# Autodesk Inventor assembly: Assembly5
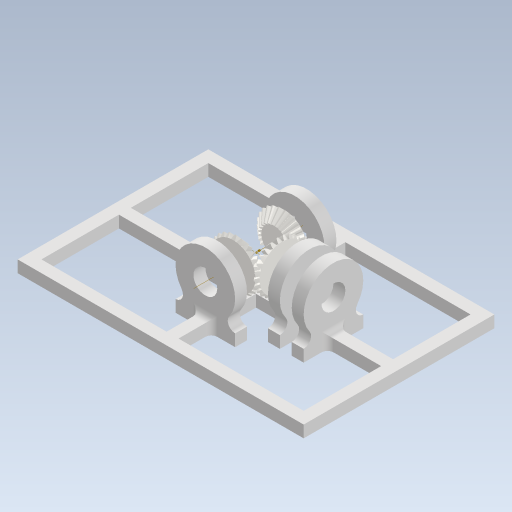
[picture p0: Inventor's stored thumbnail of the model, 512x512]
Saved by Autodesk Inventor 2023 (Build 270158000, 158)
## iProperties
Created: 2023-02-24
Part Number: Assembly5
Document SubType Name: Assembly
Designer: Dave
Author: Dave
## Documents named in this file (4)
- C:\Users\Dave\Documents\GitHub\BehrendURCMechanical\CAD\Chassis V2\Assembly5.iam
- C:\Users\Dave\Documents\GitHub\BehrendURCMechanical\CAD\Chassis V2\Chassis.ipt
- C:\Users\Dave\Documents\GitHub\BehrendURCMechanical\CAD\Chassis V2\Assembly1\Design Accelerator\Bevel Gear23.ipt
- C:\Users\Dave\Documents\GitHub\BehrendURCMechanical\CAD\Chassis V2\Assembly1\Design Accelerator\Bevel Gear13.ipt
## Components (4 placed, 3 different names)
1. Chassis:1 — Mate:1, Mate:2, Mate:3
2. Bevel Gear2:1 — Mate:2
3. Bevel Gear2:2 — Mate:3
4. Bevel Gear1:1 — Mate:1
## Relationships (3: Mate 3)
- Mate:1: Chassis:1 ↔ Bevel Gear1:1
- Mate:2: Chassis:1 ↔ Bevel Gear2:1
- Mate:3: Chassis:1 ↔ Bevel Gear2:2
